# Autodesk Inventor assembly: Positioning tool
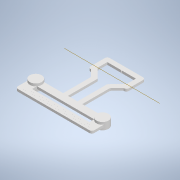
[picture p0: Inventor's stored thumbnail of the model, 180x180]
Saved by Autodesk Inventor 2021.2 (Build 252289000, 289)
## iProperties
Created: 2021-06-08
Part Number: Positioning tool
Document SubType Name: Assembly
Designer: jl4459
Author: jl4459
## Documents named in this file (4)
- C:\Users\jl4459\Documents\Inventor\VR Rigs\Modules\Positioning tool\Positioning tool mini VR.iam
- C:\Users\jl4459\Documents\Inventor\VR Rigs\Modules\Positioning tool\Parts\Positioning tool mini VR.ipt
- C:\Users\jl4459\Documents\Inventor\VR Rigs\Modules\Positioning tool\Parts\5862K163_HIGH-PULL RARE EARTH MAGNETIC DISC.ipt
- C:\Users\jl4459\Documents\Inventor\VR Rigs\Modules\Positioning tool\Parts\98535A136_1095 SPRING STEEL MACHINE KEY STOCK.ipt
## Components (4 placed, 3 different names)
1. Positioning tool mini VR:1 — Insert:1, Insert:2, Mate:1, Mate:2, Mate:3
2. 5862K163_HIGH-PULL RARE EARTH MAGNETIC DISC:1 — Insert:2
3. 5862K163_HIGH-PULL RARE EARTH MAGNETIC DISC:2 — Insert:1
4. 98535A136_1095 SPRING STEEL MACHINE KEY STOCK:1 — Mate:1, Mate:2, Mate:3
## Relationships (5: Mate 3, Insert 2)
- Insert:1: Positioning tool mini VR:1 ↔ 5862K163_HIGH-PULL RARE EARTH MAGNETIC DISC:2
- Insert:2: Positioning tool mini VR:1 ↔ 5862K163_HIGH-PULL RARE EARTH MAGNETIC DISC:1
- Mate:1: Positioning tool mini VR:1 ↔ 98535A136_1095 SPRING STEEL MACHINE KEY STOCK:1
- Mate:2: Positioning tool mini VR:1 ↔ 98535A136_1095 SPRING STEEL MACHINE KEY STOCK:1
- Mate:3: Positioning tool mini VR:1 ↔ 98535A136_1095 SPRING STEEL MACHINE KEY STOCK:1
